# Autodesk Inventor assembly: Turret Columb Assembly
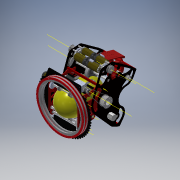
[picture p0: Inventor's stored thumbnail of the model, 180x180]
Saved by Autodesk Inventor 2019.4 (Build 234330000, 330)
## iProperties
Created: 2020-01-18
Part Number: Turret Columb Assembly
Document SubType Name: Assembly
Designer: admin
Mass: 13582.1 g
Surface Area: 21263.1 cm^2
Volume: 13067.7 cm^3
Density: 1.03936 g/cm^3
Author: admin
## Documents named in this file (24)
- C:\Users\admin\Desktop\FRC 2020 Engineering\GitHub\7738-2020\Robot V2\Turret Columb Assembly\Turret Columb Assembly.iam
- C:\Users\admin\Desktop\FRC 2020 Engineering\GitHub\7738-2020\Robot V2\Turret\Turret Assembly.iam
- C:\Users\admin\Desktop\FRC 2020 Engineering\GitHub\7738-2020\Robot V2\Turret Columb Assembly\Column Plate.ipt
- C:\Users\admin\Desktop\FRC 2020 Engineering\GitHub\7738-2020\Robot V2\Turret Columb Assembly\1001 Gearbox\VersaPlanetary_v1_Two_Stage_100_1_with_BAG.iam
- C:\Users\admin\Desktop\FRC 2020 Engineering\GitHub\7738-2020\Robot V2\Turret Columb Assembly\Turret Columb Assembly\Design Accelerator\Synchronous Belts Transmission1.iam
- C:\Users\admin\Desktop\FRC 2020 Engineering\GitHub\7738-2020\Robot V2\Turret Columb Assembly\Turret Columb Assembly\Design Accelerator\Synchronous Belts Transmission2.iam
- C:\Users\admin\Desktop\FRC 2020 Engineering\GitHub\7738-2020\Robot V2\Turret Columb Assembly\Turret Columb Assembly\Design Accelerator\Synchronous Belts Transmission3.iam
- C:\Users\admin\Desktop\FRC 2020 Engineering\GitHub\7738-2020\Robot V2\Turret Columb Assembly\Turret Columb Assembly\Design Accelerator\Synchronous Belts Transmission4.iam
- C:\Users\admin\Desktop\FRC 2020 Engineering\GitHub\7738-2020\Robot V2\Turret Columb Assembly\Bearing Plate.ipt
- C:\Users\admin\Desktop\FRC 2020 Engineering\GitHub\7738-2020\Robot V2\Turret\F6800.ipt
- C:\Users\admin\Desktop\FRC 2020 Engineering\GitHub\7738-2020\CAD\F6804zz.ipt
- C:\Users\admin\Desktop\FRC 2020 Engineering\GitHub\7738-2020\Robot V2\Turret Columb Assembly\Turret Columb Assembly\Design Accelerator\Synchronous Belts Transmission5.iam
- C:\Users\admin\Desktop\FRC 2020 Engineering\GitHub\7738-2020\Robot V2\Turret\775\775pro_775pro_Connect_and_8T_Pinion_217-6459.iam
- C:\Users\admin\Desktop\FRC 2020 Engineering\GitHub\7738-2020\Robot V2\Turret\36t_Aluminum_Spur_Gear_20_DP_1_2_Hex_Bore_217-3214.ipt
- C:\Users\admin\Desktop\FRC 2020 Engineering\GitHub\7738-2020\Robot V2\Turret Columb Assembly\Turret Columb Assembly\Design Accelerator\Synchronous Belts Transmission7.iam
- C:\Users\admin\Desktop\FRC 2020 Engineering\GitHub\7738-2020\Robot V2\Turret Columb Assembly\Column Axle.ipt
- C:\Users\admin\Desktop\FRC 2020 Engineering\GitHub\7738-2020\Robot V2\Turret Columb Assembly\Turret Idle Pin.ipt
- C:\Users\admin\Desktop\FRC 2020 Engineering\GitHub\7738-2020\Robot V2\Turret Columb Assembly\Column Mount.ipt
- C:\Users\admin\Desktop\FRC 2020 Engineering\GitHub\7738-2020\Robot V2\Turret Columb Assembly\Column Spacer.ipt
- C:\Users\admin\Desktop\FRC 2020 Engineering\GitHub\7738-2020\Robot V2\Turret Columb Assembly\Idle Drive Axle.ipt
- C:\Users\admin\Desktop\FRC 2020 Engineering\GitHub\7738-2020\Power Cell.ipt
- C:\Users\admin\Desktop\FRC 2020 Engineering\GitHub\7738-2020\Robot V2\Turret Columb Assembly\Bearing Spacer.ipt
- C:\Users\admin\Desktop\FRC 2020 Engineering\GitHub\7738-2020\Robot V2\Turret Columb Assembly\Slewing Bearing.ipt
- C:\Users\admin\Desktop\FRC 2020 Engineering\GitHub\7738-2020\Robot V2\Turret\Turret Sensor Mount.ipt
## Components (48 placed, 18 different names)
1. Turret Assembly:1 [sub-assembly] — Mate:1, Mate:4, Mate:5, Mate:6, Mate:40, Mate:42, Mate:113, Mate:116, Mate:117, Mate:119, Mate:120, Angle:4
2. Column Plate:1 — Mate:2, Mate:3, Mate:5, Mate:26, Mate:27, Mate:28, Mate:29, Mate:35, Mate:36, Mate:37, Mate:38, Mate:61, Mate:62, Flush:2, Mate:76, Flush:4, Mate:78, Mate:80, Mate:81, Mate:86, Mate:89, Mate:124
3. Column Plate:2 — Mate:2, Mate:3, Mate:4, Mate:6, Mate:20, Mate:21, Mate:23, Mate:24, Mate:25, Mate:30, Mate:31, Mate:32, Mate:33, Mate:34, Mate:41, Mate:43, Mate:45, Mate:75, Flush:3, Mate:82, Mate:83, Mate:84, Mate:85, Mate:87, Mate:88, Mate:109, Mate:110
4. VersaPlanetary_v1_Two_Stage_100_1_with_BAG:1 [sub-assembly] — Angle:3, Mate:44, Flush:2
5. Synchronous Belts Transmission:1 [sub-assembly]
6. Synchronous Belts Transmission:2 [sub-assembly]
7. Synchronous Belts Transmission:3 [sub-assembly]
8. Synchronous Belts Transmission:4 [sub-assembly] — Mate:46, Mate:48
9. Bearing Plate:1 — Mate:20, Mate:21, Flush:1, Angle:3, Mate:74, Mate:77, Mate:94, Mate:95, Mate:111, Angle:4
10. F6800:1 — Mate:23, Mate:34
11. F6800:2 — Mate:25, Mate:31, Mate:47, Mate:49, Mate:50
12. F6800:3 — Mate:24, Mate:33
13. F6800:4 — Mate:26, Mate:36
14. F6800:5 — Mate:29, Mate:37
15. F6800:6 — Mate:27, Mate:35, Mate:52, Mate:54
16. F6800:7 — Mate:30, Mate:32, Mate:51, Mate:56
17. F6800:8 — Mate:28, Mate:38, Mate:53, Mate:55
18. F6804zz:1 — Mate:41, Mate:43, Mate:58
19. F6804zz:3 — Mate:40, Mate:42, Mate:57
20. Synchronous Belts Transmission:5 [sub-assembly] — Mate:44
21. 775pro_775pro_Connect_and_8T_Pinion_217-6459:1 [sub-assembly] — Mate:45, Mate:48
22. 36t_Aluminum_Spur_Gear_20_DP_1_2_Hex_Bore_217-3214:1 — Mate:46, Mate:47
23. Synchronous Belts Transmission:6 [sub-assembly]
24. Column Axle:1 — Mate:53, Mate:55
25. Column Axle:2 — Mate:52, Mate:54
26. Column Axle:3 — Mate:51, Mate:56
27. Column Axle:4 — Mate:49, Mate:50
28. Turret Idle Pin:1 — Mate:57, Mate:58
29. F6804zz:4 — Mate:61, Mate:62, Mate:115, Flush:5
30. Column Mount:1 — Mate:74, Mate:75, Flush:3, Mate:109, Mate:110
31. Column Mount:2 — Mate:76, Mate:77, Flush:4
32. Column Spacer:1 — Mate:78, Mate:84
33. Column Spacer:2 — Mate:85, Mate:124
34. Column Spacer:3 — Mate:80, Mate:83
35. Column Spacer:4 — Mate:81, Mate:82
36. F6800:9 — Mate:86, Mate:89, Mate:90, Mate:91
37. F6800:10 — Mate:87, Mate:88
38. Idle Drive Axle:1 — Mate:90, Mate:91
39. Power Cell:1 — Mate:92
40. Bearing Spacer:1 — Mate:96, Mate:97, Mate:98, Mate:111
41. Slewing Bearing:1 — Mate:93, Mate:94, Mate:95, Mate:96, Mate:97, Mate:98, Mate:99, Mate:100, Mate:101
42. Bearing Spacer:2 — Mate:99, Mate:100, Mate:101, Mate:108, Mate:112
43. Slewing Bearing:2 — Mate:93, Mate:102, Mate:103, Mate:104, Mate:105, Mate:106, Mate:107
44. Bearing Spacer:3 — Mate:102, Mate:105, Mate:107, Mate:108, Mate:112
45. Bearing Spacer:4 — Mate:103, Mate:104, Mate:106
46. Turret Sensor Mount:1 — Mate:113, Mate:114, Mate:123
47. Turret Idle Pin:2 — Mate:115, Flush:5
48. F6804zz:5 — Mate:116, Mate:117
## Relationships (101: Mate 94, Flush 5, Angle 2)
- Mate:1: Turret Assembly:1
- Mate:2: Column Plate:1 ↔ Column Plate:2
- Mate:3: Column Plate:1 ↔ Column Plate:2
- Mate:4 (5 mm): Turret Assembly:1 ↔ Column Plate:2
- Mate:5 (5 mm): Turret Assembly:1 ↔ Column Plate:1
- Mate:6: Turret Assembly:1 ↔ Column Plate:2
- Mate:20 (1 mm): Column Plate:2 ↔ Bearing Plate:1
- Mate:21 (1 mm): Column Plate:2 ↔ Bearing Plate:1
- Flush:1 (21 mm): Bearing Plate:1
- Mate:23: Column Plate:2 ↔ F6800:1
- Mate:24: Column Plate:2 ↔ F6800:3
- Mate:25: Column Plate:2 ↔ F6800:2
- Mate:26: Column Plate:1 ↔ F6800:4
- Mate:27: Column Plate:1 ↔ F6800:6
- Mate:28: Column Plate:1 ↔ F6800:8
- Mate:29: Column Plate:1 ↔ F6800:5
- Mate:30: Column Plate:2 ↔ F6800:7
- Mate:31 (0.2 mm): Column Plate:2 ↔ F6800:2
- Mate:32 (0.2 mm): Column Plate:2 ↔ F6800:7
- Mate:33 (0.2 mm): Column Plate:2 ↔ F6800:3
- Mate:34 (0.2 mm): Column Plate:2 ↔ F6800:1
- Mate:35 (0.2 mm): Column Plate:1 ↔ F6800:6
- Mate:36 (0.2 mm): Column Plate:1 ↔ F6800:4
- Mate:37 (0.2 mm): Column Plate:1 ↔ F6800:5
- Mate:38 (0.2 mm): Column Plate:1 ↔ F6800:8
- Angle:3 (0 deg): VersaPlanetary_v1_Two_Stage_100_1_with_BAG:1 ↔ Bearing Plate:1
- Mate:40: Turret Assembly:1 ↔ F6804zz:3
- Mate:41: Column Plate:2 ↔ F6804zz:1
- Mate:42 (0.2 mm): Turret Assembly:1 ↔ F6804zz:3
- Mate:43 (0.2 mm): Column Plate:2 ↔ F6804zz:1
- Mate:44: VersaPlanetary_v1_Two_Stage_100_1_with_BAG:1 ↔ Synchronous Belts Transmission:5
- Mate:45: Column Plate:2 ↔ 775pro_775pro_Connect_and_8T_Pinion_217-6459:1
- Mate:46: Synchronous Belts Transmission:4 ↔ 36t_Aluminum_Spur_Gear_20_DP_1_2_Hex_Bore_217-3214:1
- Mate:47 (2 mm): F6800:2 ↔ 36t_Aluminum_Spur_Gear_20_DP_1_2_Hex_Bore_217-3214:1
- Mate:48 (29.21 mm): Synchronous Belts Transmission:4 ↔ 775pro_775pro_Connect_and_8T_Pinion_217-6459:1
- Mate:49: F6800:2 ↔ Column Axle:4
- Mate:50 (0.1 mm): F6800:2 ↔ Column Axle:4
- Mate:51: F6800:7 ↔ Column Axle:3
- Mate:52: F6800:6 ↔ Column Axle:2
- Mate:53: F6800:8 ↔ Column Axle:1
- Mate:54 (0.1 mm): F6800:6 ↔ Column Axle:2
- Mate:55 (0.1 mm): F6800:8 ↔ Column Axle:1
- Mate:56 (0.1 mm): F6800:7 ↔ Column Axle:3
- Mate:57: F6804zz:3 ↔ Turret Idle Pin:1
- Mate:58: F6804zz:1 ↔ Turret Idle Pin:1
- Mate:61: Column Plate:1 ↔ F6804zz:4
- Mate:62 (0.2 mm): Column Plate:1 ↔ F6804zz:4
- Flush:2 (-6 mm): Column Plate:1 ↔ VersaPlanetary_v1_Two_Stage_100_1_with_BAG:1
- Mate:74: Bearing Plate:1 ↔ Column Mount:1
- Mate:75: Column Plate:2 ↔ Column Mount:1
- Flush:3 (30 mm): Column Plate:2 ↔ Column Mount:1
- Mate:76: Column Plate:1 ↔ Column Mount:2
- Mate:77: Bearing Plate:1 ↔ Column Mount:2
- Flush:4 (30 mm): Column Plate:1 ↔ Column Mount:2
- Mate:78: Column Plate:1 ↔ Column Spacer:1
- Mate:80: Column Plate:1 ↔ Column Spacer:3
- Mate:81: Column Plate:1 ↔ Column Spacer:4
- Mate:82: Column Plate:2 ↔ Column Spacer:4
- Mate:83: Column Plate:2 ↔ Column Spacer:3
- Mate:84: Column Plate:2 ↔ Column Spacer:1
- Mate:85: Column Plate:2 ↔ Column Spacer:2
- Mate:86: Column Plate:1 ↔ F6800:9
- Mate:87: Column Plate:2 ↔ F6800:10
- Mate:88 (0.2 mm): Column Plate:2 ↔ F6800:10
- Mate:89 (0.2 mm): Column Plate:1 ↔ F6800:9
- Mate:90: F6800:9 ↔ Idle Drive Axle:1
- Mate:91: F6800:9 ↔ Idle Drive Axle:1
- Mate:92: Power Cell:1
- Mate:93: Slewing Bearing:1 ↔ Slewing Bearing:2
- Mate:94: Bearing Plate:1 ↔ Slewing Bearing:1
- Mate:95: Bearing Plate:1 ↔ Slewing Bearing:1
- Mate:96: Bearing Spacer:1 ↔ Slewing Bearing:1
- Mate:97: Bearing Spacer:1 ↔ Slewing Bearing:1
- Mate:98: Bearing Spacer:1 ↔ Slewing Bearing:1
- Mate:99: Slewing Bearing:1 ↔ Bearing Spacer:2
- Mate:100: Slewing Bearing:1 ↔ Bearing Spacer:2
- Mate:101: Slewing Bearing:1 ↔ Bearing Spacer:2
- Mate:102: Slewing Bearing:2 ↔ Bearing Spacer:3
- Mate:103: Slewing Bearing:2 ↔ Bearing Spacer:4
- Mate:104: Slewing Bearing:2 ↔ Bearing Spacer:4
- Mate:105: Slewing Bearing:2 ↔ Bearing Spacer:3
- Mate:106: Slewing Bearing:2 ↔ Bearing Spacer:4
- Mate:107: Slewing Bearing:2 ↔ Bearing Spacer:3
- Mate:108 (5.2 mm): Bearing Spacer:2 ↔ Bearing Spacer:3
- Mate:109: Column Plate:2 ↔ Column Mount:1
- Mate:110: Column Plate:2 ↔ Column Mount:1
- Mate:111: Bearing Plate:1 ↔ Bearing Spacer:1
- Mate:112: Bearing Spacer:2 ↔ Bearing Spacer:3
- Mate:113: Turret Assembly:1 ↔ Turret Sensor Mount:1
- Mate:114 (-15 mm): Turret Sensor Mount:1
- Mate:115: F6804zz:4 ↔ Turret Idle Pin:2
- Flush:5: F6804zz:4 ↔ Turret Idle Pin:2
- Mate:116: Turret Assembly:1 ↔ F6804zz:5
- Mate:117: Turret Assembly:1 ↔ F6804zz:5
- Mate:119: Turret Assembly:1
- Mate:120: Turret Assembly:1
- Mate:121
- Mate:122
- Mate:123: Turret Sensor Mount:1
- Mate:124: Column Plate:1 ↔ Column Spacer:2
- Angle:4 (200 deg): Turret Assembly:1 ↔ Bearing Plate:1
